# Autodesk Inventor assembly: 64-106_Horn_Set
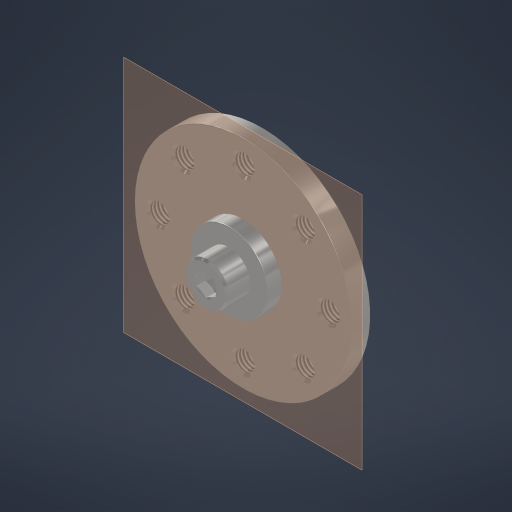
[picture p0: Inventor's stored thumbnail of the model, 512x512]
Saved by Autodesk Inventor 2024 (Build 280153000, 153)
## iProperties
Created: 2024-02-15
Part Number: 64-106_Horn_Set
Document SubType Name: Assembly
Designer: ASUS
Author: ASUS
## Documents named in this file (3)
- C:\Users\ASUS\Desktop\Anti_Backlash_Structure_OP\ROBOTIS(Inventor 2024 ver.)\혼\64-106_Horn_Set.iam
- C:\Users\ASUS\Desktop\Anti_Backlash_Structure_OP\MISUMI\CSH-STN-M3-10_203.ipt
- C:\Users\ASUS\Desktop\Anti_Backlash_Structure_OP\ROBOTIS(Inventor 2024 ver.)\혼\64-106Horn.ipt
## Components (2 placed, 2 different names)
1. CSH-STN-M3-10_203:1 — 삽입:1
2. 64-106Horn:1 — 삽입:1
## Relationships (1: Insert 1)
- 삽입:1 [Insert]: CSH-STN-M3-10_203:1 ↔ 64-106Horn:1
